# Autodesk Inventor assembly: FULL
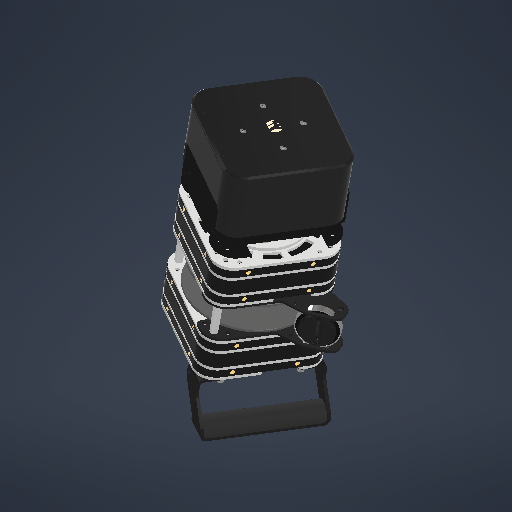
[picture p0: Inventor's stored thumbnail of the model, 512x512]
Saved by Autodesk Inventor 2026.1 (Build 301233000, 233)
## iProperties
Created: 2025-03-02
Part Number: FULL
Document SubType Name: Assembly
Designer: aaron
Author: aaron
## Documents named in this file (4)
- D:\work\loopandpixel\openworkoutsystem\cad\v5\FULL.iam
- D:\work\loopandpixel\openworkoutsystem\cad\v5\drivetrain.iam
- D:\work\loopandpixel\openworkoutsystem\cad\v5\battery_pack_16s.ipt.iam
- battery_pack_16s.ipt
## Components (2 placed, 2 different names)
1. battery_pack_16s.ipt:1 [sub-assembly] — Flush:1, Flush:2, Mate:1
2. drivetrain:2 [sub-assembly] — Flush:1, Flush:2, Mate:1
## Relationships (3: Flush 2, Mate 1)
- Flush:1: battery_pack_16s.ipt:1 ↔ drivetrain:2
- Flush:2: battery_pack_16s.ipt:1 ↔ drivetrain:2
- Mate:1: battery_pack_16s.ipt:1 ↔ drivetrain:2
